# Autodesk Inventor assembly: Cook-Assembly
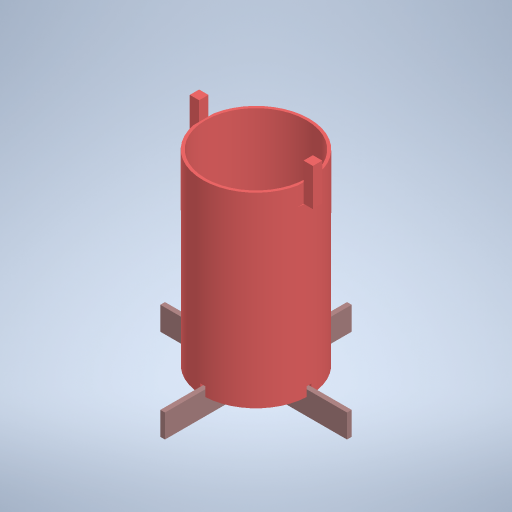
[picture p0: Inventor's stored thumbnail of the model, 512x512]
Saved by Autodesk Inventor 2024.3 (Build 283343000, 343)
## iProperties
Created: 2025-03-01
Part Number: Cook-Assembly
Document SubType Name: Assembly
Designer: ajclo
Author: ajclo
## Documents named in this file (3)
- C:\Users\ajclo\OneDrive - Stellenbosch University\Documents\BEng\Year IV\Skripsie\CAD\Cook-Assembly.iam
- C:\Users\ajclo\OneDrive - Stellenbosch University\Documents\BEng\Year IV\Skripsie\CAD\Cooking Pipe.ipt
- C:\Users\ajclo\OneDrive - Stellenbosch University\Documents\BEng\Year IV\Skripsie\CAD\PotStand.ipt
## Components (3 placed, 2 different names)
1. Cooking Pipe:1 — Mate:4, Mate:5
2. PotStand:1 — Mate:1, Mate:2, Mate:3, Mate:4
3. PotStand:2 — Mate:1, Mate:2, Mate:3, Mate:5
## Relationships (5: Mate 5)
- Mate:1: PotStand:1 ↔ PotStand:2
- Mate:2: PotStand:1 ↔ PotStand:2
- Mate:3: PotStand:1 ↔ PotStand:2
- Mate:4: Cooking Pipe:1 ↔ PotStand:1
- Mate:5: Cooking Pipe:1 ↔ PotStand:2
